# Autodesk Inventor assembly: 99550c01
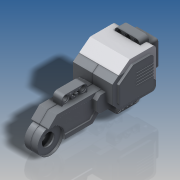
[picture p0: Inventor's stored thumbnail of the model, 180x180]
Saved by Autodesk Inventor 2016 SP2 (Build 200236200, 236)
## iProperties
Created: 2015-09-01
Part Number: 99550c01
Document SubType Name: Assembly
Designer: D. Kohfeld
Mass: 22.2612 g
Surface Area: 332.07 cm^2
Volume: 21.0012 cm^3
Density: 1.06 g/cm^3
Author: D. Kohfeld
## Documents named in this file (6)
- A:\LEGO Pieces\EV3\99550c01.iam
- A:\LEGO Pieces\EV3\99550-LtBluishGray.ipt
- A:\LEGO Pieces\EV3\99551-LtBluishGray.ipt
- A:\LEGO Pieces\EV3\10825-LtBluishGray.ipt
- A:\LEGO Pieces\EV3\99555-White.ipt
- A:\LEGO Pieces\EV3\54732b-LtBluishGray.ipt
## Components (5 placed, 5 different names)
1. 99550-LtBluishGray:1 — Mate:1, Flush:1, Flush:2, Flush:3, Flush:4, Mate:2, Flush:8
2. 99551-LtBluishGray:1 — Mate:1, Flush:1, Flush:2
3. 10825-LtBluishGray:1 — Flush:5, Mate:3, Flush:7, Mate:4, Flush:8
4. 99555-White:1 — Flush:3, Flush:4, Mate:2, Flush:6, Flush:5, Mate:4
5. 54732b-LtBluishGray:1 — Flush:6, Mate:3, Flush:7
## Relationships (12: Flush 8, Mate 4)
- Mate:1: 99550-LtBluishGray:1 ↔ 99551-LtBluishGray:1
- Flush:1: 99550-LtBluishGray:1 ↔ 99551-LtBluishGray:1
- Flush:2: 99550-LtBluishGray:1 ↔ 99551-LtBluishGray:1
- Flush:3: 99550-LtBluishGray:1 ↔ 99555-White:1
- Flush:4: 99550-LtBluishGray:1 ↔ 99555-White:1
- Mate:2: 99550-LtBluishGray:1 ↔ 99555-White:1
- Flush:6: 99555-White:1 ↔ 54732b-LtBluishGray:1
- Flush:5: 10825-LtBluishGray:1 ↔ 99555-White:1
- Mate:3: 10825-LtBluishGray:1 ↔ 54732b-LtBluishGray:1
- Flush:7: 10825-LtBluishGray:1 ↔ 54732b-LtBluishGray:1
- Mate:4: 10825-LtBluishGray:1 ↔ 99555-White:1
- Flush:8: 99550-LtBluishGray:1 ↔ 10825-LtBluishGray:1
